# Autodesk Inventor assembly: Foot
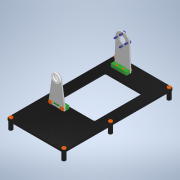
[picture p0: Inventor's stored thumbnail of the model, 180x180]
Saved by Autodesk Inventor 2020 (Build 240168000, 168)
## iProperties
Created: 2021-10-01
Part Number: Foot
Document SubType Name: Assembly
Designer: Masato Kubotera
Author: Masato Kubotera
## Documents named in this file (10)
- C:\Users\Masato\Desktop\OpenPlatform_ver3_0 - Ver4_1branch\LowerBody\Foot\Foot.iam
- C:\Users\Masato\Desktop\OpenPlatform_ver3_0 - Ver4_1branch\Ready_Made\ARU-313SMO.ipt
- C:\Users\Masato\Desktop\OpenPlatform_ver3_0 - Ver4_1branch\LowerBody\Foot\Foot_back_frame.ipt
- C:\Users\Masato\Desktop\OpenPlatform_ver3_0 - Ver4_1branch\LowerBody\Foot\Foot_front_frame.ipt
- C:\Users\Masato\Desktop\OpenPlatform_ver3_0 - Ver4_1branch\LowerBody\Foot\Foot_root_block.ipt
- C:\Users\Masato\Desktop\OpenPlatform_ver3_0 - Ver4_1branch\LowerBody\Foot\Sole_frame.ipt
- C:\Users\Masato\Desktop\OpenPlatform_ver3_0 - Ver4_1branch\Ready_Made\Screw\M3-8.ipt
- C:\Users\Masato\Desktop\OpenPlatform_ver3_0 - Ver4_1branch\Ready_Made\Screw\M3-6.ipt
- C:\Users\Masato\Desktop\OpenPlatform_ver3_0 - Ver4_1branch\Ready_Made\TT-0814-15.ipt
- C:\Users\Masato\Desktop\OpenPlatform_ver3_0 - Ver4_1branch\Ready_Made\Screw\M2_6-6.ipt
## Components (30 placed, 9 different names)
1. ARU-313SMO:1 — 挿入:6
2. ARU-313SMO:2 — 挿入:5
3. ARU-313SMO:3 — 挿入:4
4. ARU-313SMO:4 — 挿入:3
5. ARU-313SMO:5 — 挿入:2
6. ARU-313SMO:6 — 挿入:1
7. Foot_back_frame:1 — 挿入:11, 挿入:12, 挿入:25, 挿入:26, 挿入:35, 挿入:36, 挿入:37, 挿入:38
8. Foot_front_frame:1 — 挿入:13, 挿入:14, 挿入:23, 挿入:24, メイト:2, 挿入:31
9. Foot_root_block:1 — 挿入:7, 挿入:8, 挿入:13, 挿入:14
10. Foot_root_block:2 — 挿入:9, 挿入:10, 挿入:11, 挿入:12
11. Sole_frame:1 — メイト:1, フラッシュ:1, 挿入:1, 挿入:2, 挿入:3, 挿入:4, 挿入:5, 挿入:6, 挿入:7, 挿入:8, 挿入:9, 挿入:10, 挿入:17, 挿入:18, 挿入:19, 挿入:20, 挿入:21, 挿入:22, 挿入:27, 挿入:28, 挿入:29, 挿入:30
12. M3-8:1 — 挿入:17
13. M3-8:2 — 挿入:18
14. M3-8:3 — 挿入:19
15. M3-8:4 — 挿入:20
16. M3-8:5 — 挿入:21
17. M3-8:6 — 挿入:22
18. M3-6:1 — 挿入:23
19. M3-6:2 — 挿入:24
20. M3-6:3 — 挿入:26
21. M3-6:4 — 挿入:25
22. M3-8:7 — 挿入:27
23. M3-8:8 — 挿入:28
24. M3-8:9 — 挿入:29
25. M3-8:10 — 挿入:30
26. TT-0814-15:1 — 挿入:31
27. M2_6-6:1 — 挿入:35
28. M2_6-6:2 — 挿入:36
29. M2_6-6:3 — 挿入:37
30. M2_6-6:4 — 挿入:38
## Relationships (36: Insert 33, Mate 2, Flush 1)
- メイト:1 [Mate]: Sole_frame:1
- フラッシュ:1 [Flush]: Sole_frame:1
- 挿入:1 [Insert]: ARU-313SMO:6 ↔ Sole_frame:1
- 挿入:2 [Insert]: ARU-313SMO:5 ↔ Sole_frame:1
- 挿入:3 [Insert]: ARU-313SMO:4 ↔ Sole_frame:1
- 挿入:4 [Insert]: ARU-313SMO:3 ↔ Sole_frame:1
- 挿入:5 [Insert]: ARU-313SMO:2 ↔ Sole_frame:1
- 挿入:6 [Insert]: ARU-313SMO:1 ↔ Sole_frame:1
- 挿入:7 [Insert]: Foot_root_block:1 ↔ Sole_frame:1
- 挿入:8 [Insert]: Foot_root_block:1 ↔ Sole_frame:1
- 挿入:9 [Insert]: Foot_root_block:2 ↔ Sole_frame:1
- 挿入:10 [Insert]: Foot_root_block:2 ↔ Sole_frame:1
- 挿入:11 [Insert]: Foot_back_frame:1 ↔ Foot_root_block:2
- 挿入:12 [Insert]: Foot_back_frame:1 ↔ Foot_root_block:2
- 挿入:13 [Insert]: Foot_front_frame:1 ↔ Foot_root_block:1
- 挿入:14 [Insert]: Foot_front_frame:1 ↔ Foot_root_block:1
- 挿入:17 [Insert]: Sole_frame:1 ↔ M3-8:1
- 挿入:18 [Insert]: Sole_frame:1 ↔ M3-8:2
- 挿入:19 [Insert]: Sole_frame:1 ↔ M3-8:3
- 挿入:20 [Insert]: Sole_frame:1 ↔ M3-8:4
- 挿入:21 [Insert]: Sole_frame:1 ↔ M3-8:5
- 挿入:22 [Insert]: Sole_frame:1 ↔ M3-8:6
- 挿入:23 [Insert]: Foot_front_frame:1 ↔ M3-6:1
- 挿入:24 [Insert]: Foot_front_frame:1 ↔ M3-6:2
- 挿入:25 [Insert]: Foot_back_frame:1 ↔ M3-6:4
- 挿入:26 [Insert]: Foot_back_frame:1 ↔ M3-6:3
- メイト:2 [Mate]: Foot_front_frame:1
- 挿入:27 [Insert]: Sole_frame:1 ↔ M3-8:7
- 挿入:28 [Insert]: Sole_frame:1 ↔ M3-8:8
- 挿入:29 [Insert]: Sole_frame:1 ↔ M3-8:9
- 挿入:30 [Insert]: Sole_frame:1 ↔ M3-8:10
- 挿入:31 [Insert]: Foot_front_frame:1 ↔ TT-0814-15:1
- 挿入:35 [Insert]: Foot_back_frame:1 ↔ M2_6-6:1
- 挿入:36 [Insert]: Foot_back_frame:1 ↔ M2_6-6:2
- 挿入:37 [Insert]: Foot_back_frame:1 ↔ M2_6-6:3
- 挿入:38 [Insert]: Foot_back_frame:1 ↔ M2_6-6:4
